# Autodesk Inventor assembly: XY Drive Subassy
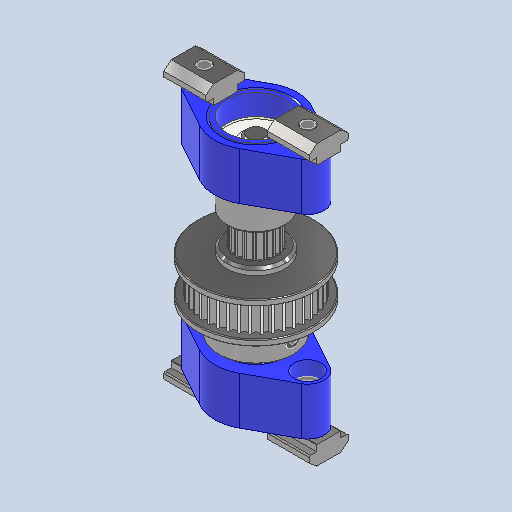
[picture p0: Inventor's stored thumbnail of the model, 512x512]
Saved by Autodesk Inventor 2022 (Build 260153000, 153)
## iProperties
Created: 2021-10-06
Part Number: XY Drive Subassy
Document SubType Name: Assembly
Designer: nicol
Author: nicol
## Documents named in this file (10)
- Y:\Projects\Bibble0\SubAsm\XY Drive Subassy.iam
- Y:\Projects\Bibble0\Bearings\625 Bearing.ipt
- Y:\Projects\Bibble0\3D printed\X-Y Axis\XY Drive Bearing Holder.ipt
- Y:\Projects\Bibble0\Hardware\GT2 Pulley 16T.ipt
- Y:\Projects\Bibble0\Hardware\5 x 50mm Shaft.ipt
- Y:\Projects\Bibble0\3D printed\X-Y Axis\Bearing Retaining Ring.ipt
- Y:\Projects\Bibble0\Hardware\GT2 40T 5mm Bore.ipt
- Y:\Projects\Bibble0\3D printed\5mmx3mm spacer.ipt
- Y:\Projects\Bibble0\Hardware\M3 x 10 mm SHCS.ipt
- Y:\Projects\Bibble0\Hardware\M3 T-Slot Nut.ipt
## Components (19 placed, 9 different names)
1. 625 Bearing:1 — Insert:7, Insert:13, Insert:15, Insert:16
2. 625 Bearing:2 — Insert:8, Insert:11, Insert:14
3. XY Drive Bearing Holder:1 — Mate:1, Insert:14, Insert:19, Insert:20, Insert:21, Insert:22, Angle:2
4. XY Drive Bearing Holder:2 — Mate:1, Insert:15, Insert:17, Insert:18, Insert:23, Insert:24
5. GT2 Pulley 16T:2 — Insert:9, Insert:10
6. 5 x 50mm Shaft:1 — Insert:16
7. Bearing Retaining Ring:1 — Insert:7
8. Bearing Retaining Ring:2 — Insert:8
9. GT2 40T 5mm Bore:1 — Insert:9, Insert:12
10. 5mmx3mm spacer:1 — Insert:10, Insert:11
11. 5mmx3mm spacer:2 — Insert:12, Insert:13
12. M3 x 10 mm SHCS:1 — Insert:17
13. M3 x 10 mm SHCS:2 — Insert:18
14. M3 x 10 mm SHCS:3 — Insert:19
15. M3 x 10 mm SHCS:4 — Insert:20
16. M3 T-Slot Nut:1 — Insert:21, Angle:3
17. M3 T-Slot Nut:2 — Insert:22, Angle:3, Angle:4
18. M3 T-Slot Nut:3 — Insert:23, Angle:1
19. M3 T-Slot Nut:4 — Insert:24, Angle:1, Angle:5
## Relationships (24: Insert 18, Angle 5, Mate 1)
- Insert:7: 625 Bearing:1 ↔ Bearing Retaining Ring:1
- Insert:8: 625 Bearing:2 ↔ Bearing Retaining Ring:2
- Mate:1: XY Drive Bearing Holder:1 ↔ XY Drive Bearing Holder:2
- Insert:9: GT2 Pulley 16T:2 ↔ GT2 40T 5mm Bore:1
- Insert:10: GT2 Pulley 16T:2 ↔ 5mmx3mm spacer:1
- Insert:11: 625 Bearing:2 ↔ 5mmx3mm spacer:1
- Insert:12: GT2 40T 5mm Bore:1 ↔ 5mmx3mm spacer:2
- Insert:13: 625 Bearing:1 ↔ 5mmx3mm spacer:2
- Insert:14: 625 Bearing:2 ↔ XY Drive Bearing Holder:1
- Insert:15: 625 Bearing:1 ↔ XY Drive Bearing Holder:2
- Insert:16: 625 Bearing:1 ↔ 5 x 50mm Shaft:1
- Insert:17: XY Drive Bearing Holder:2 ↔ M3 x 10 mm SHCS:1
- Insert:18: XY Drive Bearing Holder:2 ↔ M3 x 10 mm SHCS:2
- Insert:19: XY Drive Bearing Holder:1 ↔ M3 x 10 mm SHCS:3
- Insert:20: XY Drive Bearing Holder:1 ↔ M3 x 10 mm SHCS:4
- Insert:21: XY Drive Bearing Holder:1 ↔ M3 T-Slot Nut:1
- Insert:22: XY Drive Bearing Holder:1 ↔ M3 T-Slot Nut:2
- Insert:23: XY Drive Bearing Holder:2 ↔ M3 T-Slot Nut:3
- Insert:24: XY Drive Bearing Holder:2 ↔ M3 T-Slot Nut:4
- Angle:1 (180 deg): M3 T-Slot Nut:3 ↔ M3 T-Slot Nut:4
- Angle:2 (0 deg): XY Drive Bearing Holder:1
- Angle:3 (0 deg): M3 T-Slot Nut:1 ↔ M3 T-Slot Nut:2
- Angle:4 (0 deg): M3 T-Slot Nut:2
- Angle:5 (0 deg): M3 T-Slot Nut:4
